# Autodesk Inventor assembly: 276-2010
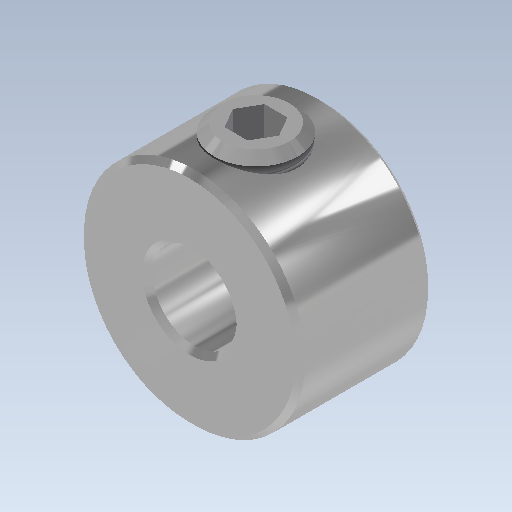
[picture p0: Inventor's stored thumbnail of the model, 512x512]
Saved by Autodesk Inventor 2020.2 (Build 242310000, 310)
## iProperties
Created: 2012-04-11
Document SubType Name: Assembly
Designer: Autodesk Inc.
Part Number: 276-2010
Catalog Web Link: http://www.vexrobotics.com/276-2010.html
Vendor: VEX
Company: Autodesk Inc.
Category: Motion
Author: Autodesk Inc.
## Documents named in this file (3)
- C:\Users\vedag\Documents\GitHub\VEX-90819\VRC 2019-2020 Tower Takeover\Inventor Files\Motion\Shafts and Related\Shaft Collar.iam
- C:\Users\vedag\Documents\GitHub\VEX-90819\VRC 2019-2020 Tower Takeover\Inventor Files\Motion\Components\Shaft Collar.ipt
- C:\Users\vedag\Documents\GitHub\VEX-90819\VRC 2019-2020 Tower Takeover\Inventor Files\Motion\Components\ANSI B18.3 - 8-32 UNC - 0.1875(32)306.ipt
## Components (2 placed, 2 different names)
1. Shaft Collar:1 — Mate:1, Flush:1, Angle:1
2. Type B - Hexagon Socket Set Screw - Cup Point - Inch 8-32 UNC - 0.1875:1 — Mate:1, Flush:1, Angle:1
## Relationships (3: Mate 1, Flush 1, Angle 1)
- Mate:1: Shaft Collar:1 ↔ Type B - Hexagon Socket Set Screw - Cup Point - Inch 8-32 UNC - 0.1875:1
- Flush:1 (-0.508 mm): Shaft Collar:1 ↔ Type B - Hexagon Socket Set Screw - Cup Point - Inch 8-32 UNC - 0.1875:1
- Angle:1 (0 deg): Shaft Collar:1 ↔ Type B - Hexagon Socket Set Screw - Cup Point - Inch 8-32 UNC - 0.1875:1
